# Autodesk Inventor assembly: arm
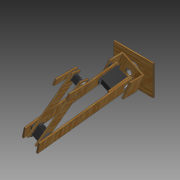
[picture p0: Inventor's stored thumbnail of the model, 180x180]
Saved by Autodesk Inventor 2013 (Build 170138000, 138)
## iProperties
Created: 2014-10-10
Part Number: arm
Document SubType Name: Assembly
Designer: Masta
Author: Masta
## Documents named in this file (6)
- D:\DrOctopus\3D model\arm.iam
- D:\DrOctopus\3D model\segment1.iam
- D:\DrOctopus\3D model\segment2.iam
- D:\DrOctopus\3D model\segment0.iam
- D:\DrOctopus\3D model\segment3.iam
- D:\DrOctopus\3D model\base.iam
## Components (5 placed, 5 different names)
1. segment1:1 [sub-assembly] — Insert:1, Insert:2, Angle:1, Angle:2
2. segment2:1 [sub-assembly] — Insert:1, Angle:1, Insert:3
3. segment0:1 [sub-assembly] — Insert:2, Angle:2, Insert:4, Angle:3
4. segment3:1 [sub-assembly] — Insert:3, Angle:4
5. base:1 [sub-assembly] — Mate:1, Mate:2, Insert:4, Mate:3, Angle:3
## Relationships (11: Insert 4, Angle 4, Mate 3)
- Insert:1: segment1:1 ↔ segment2:1
- Insert:2: segment1:1 ↔ segment0:1
- Angle:1 (30 deg): segment1:1 ↔ segment2:1
- Angle:2 (45 deg): segment1:1 ↔ segment0:1
- Insert:3: segment2:1 ↔ segment3:1
- Mate:1: base:1
- Mate:2: base:1
- Insert:4 (1 mm): segment0:1 ↔ base:1
- Mate:3: base:1
- Angle:3 (0 deg): segment0:1 ↔ base:1
- Angle:4 (0 deg): segment3:1
